# Autodesk Inventor assembly: Spin-Chuck Slide
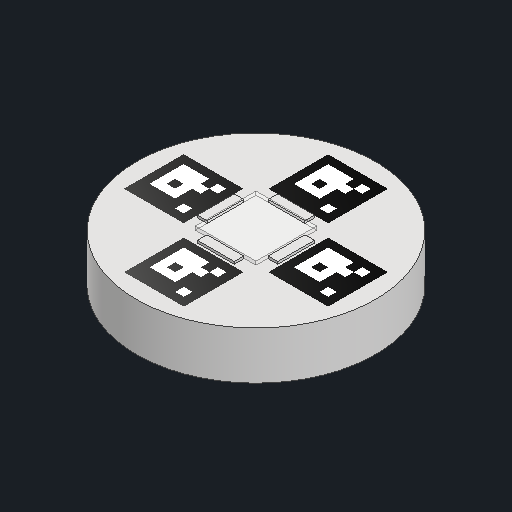
[picture p0: Inventor's stored thumbnail of the model, 512x512]
Saved by Autodesk Inventor 2025.1 (Build 291241000, 241)
## iProperties
Created: 2024-11-17
Part Number: Spin-Chuck Slide
Document SubType Name: Assembly
Designer: jerem
Author: jerem
## Documents named in this file (3)
- C:\Users\jerem\Documents\GitHub\Perovskite-Automated-Synthesis-System\CAD\Spin-Chuck\Spin-Chuck Slide.iam
- C:\Users\jerem\Documents\GitHub\Perovskite-Automated-Synthesis-System\CAD\Spin-Chuck\Spin Chuck.ipt
- C:\Users\jerem\Documents\GitHub\Perovskite-Automated-Synthesis-System\CAD\Non 3D Printed Parts\Objects\Glass Slide.ipt
## Components (2 placed, 2 different names)
1. Spin Chuck:1 — Mate:1, Mate:2, Mate:3
2. Glass Slide:1 — Mate:1, Mate:2, Mate:3
## Relationships (3: Mate 3)
- Mate:1: Spin Chuck:1 ↔ Glass Slide:1
- Mate:2: Spin Chuck:1 ↔ Glass Slide:1
- Mate:3: Spin Chuck:1 ↔ Glass Slide:1
